# Autodesk Inventor assembly: main_assembly
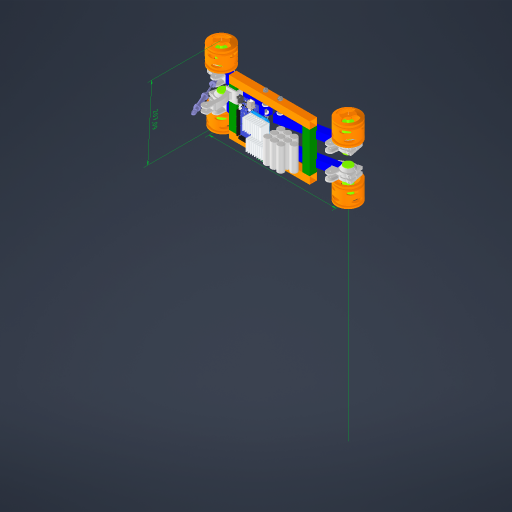
[picture p0: Inventor's stored thumbnail of the model, 512x512]
Saved by Autodesk Inventor 2024 (Build 280153000, 153)
## iProperties
Created: 2023-09-26
Part Number: main_assembly
Document SubType Name: Assembly
Designer: user
Author: user
## Documents named in this file (9)
- D:\Docs\Robot\3d_v2\main_assembly.iam
- D:\Docs\Robot\3d_v2\base\base_assambly.iam
- D:\Docs\Robot\3d_v2\machine_body\arm_assembly_r.iam
- D:\Docs\Robot\3d_v2\machine_body\arm_assembly_l.iam
- D:\Docs\Robot\3d_v2\default_components\shock_absorber.ipt
- D:\Docs\Robot\3d_v2\electronics\Battery_18650_asembly.iam
- D:\Docs\Robot\3d_v2\electronics\Arduino MEGA 2560 R3.ipt
- D:\Docs\Robot\3d_v2\electronics\BTS7960\BTS7960.iam
- D:\Docs\Robot\3d_v2\machine_body\shok_absorber_holder.ipt
## Components (12 placed, 8 different names)
1. base_assambly:1 [sub-assembly] — Совмещение:1, Совмещение:2, Совмещение:3, Вставка:1, Вставка:2, Вставка:4, Вставка:5, Совмещение:4, Совмещение:5
2. arm_assembly_r:1 [sub-assembly] — Вставка:1
3. arm_assembly_l:1 [sub-assembly] — Вставка:2, Вставка:3
4. shock_absorber:1 — Вставка:3
5. arm_assembly_l:2 [sub-assembly] — Вставка:5
6. arm_assembly_r:2 [sub-assembly] — Вставка:4
7. Battery_18650_asembly:1 [sub-assembly]
8. Arduino MEGA 2560 R3:1
9. BTS7960:1 [sub-assembly]
10. BTS7960:2 [sub-assembly]
11. shok_absorber_holder:1 — Совмещение:4, Совмещение:5
12. arm_assembly_r:3 [sub-assembly]
## Relationships (10: Mate 5, Insert 5)
- Совмещение:1 [Mate]: base_assambly:1
- Совмещение:2 [Mate]: base_assambly:1
- Совмещение:3 [Mate]: base_assambly:1
- Вставка:1 [Insert]: base_assambly:1 ↔ arm_assembly_r:1
- Вставка:2 [Insert]: base_assambly:1 ↔ arm_assembly_l:1
- Вставка:3 [Insert]: arm_assembly_l:1 ↔ shock_absorber:1
- Вставка:4 [Insert]: base_assambly:1 ↔ arm_assembly_r:2
- Вставка:5 [Insert]: base_assambly:1 ↔ arm_assembly_l:2
- Совмещение:4 [Mate]: base_assambly:1 ↔ shok_absorber_holder:1
- Совмещение:5 [Mate]: base_assambly:1 ↔ shok_absorber_holder:1
